# Autodesk Inventor assembly: 付け根_1
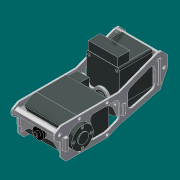
[picture p0: Inventor's stored thumbnail of the model, 180x180]
Saved by Autodesk Inventor 2016 (Build 200138000, 138)
## iProperties
Created: 2016-04-27
Part Number: 付け根_1
Document SubType Name: Assembly
Designer: hiroaki
Mass: 228.077 g
Surface Area: 379.105 cm^2
Volume: 115.513 cm^3
Density: 1.97447 g/cm^3
Author: hiroaki
## Documents named in this file (12)
- C:\Users\hiro\Documents\kenkyuu\二足\二足ver6.0\下半身\足首\足首_1.iam
- C:\Users\hiro\Documents\kenkyuu\二足\二足ver6.0\既製品\B3M11xx.ipt
- C:\Users\hiro\Documents\kenkyuu\二足\二足ver6.0\既製品\free_horn.ipt
- C:\Users\hiro\Documents\kenkyuu\二足\二足ver6.0\下半身\足首\足首_メインフレーム_1_1.ipt
- C:\Users\hiro\Documents\kenkyuu\二足\二足ver6.0\下半身\足首\足首_サブフレーム_1_1.ipt
- C:\Users\hiro\Documents\kenkyuu\二足\二足ver6.0\下半身\足首\足首_サブフレーム_1_2.ipt
- C:\Users\hiro\Documents\kenkyuu\二足\二足ver6.0\下半身\足首\足首_メインフレーム_1_1_MIR.ipt
- C:\Users\hiro\Documents\kenkyuu\二足\二足ver6.0\下半身\足首\足首_サブフレーム_1_3.ipt
- C:\Users\hiro\Documents\kenkyuu\二足\二足ver6.0\下半身\足裏\足裏_サブフレーム_1_2.ipt
- C:\Users\hiro\Documents\kenkyuu\二足\二足ver6.0\既製品\B3M10xx.ipt
- C:\Users\hiro\Documents\kenkyuu\二足\二足ver6.0\既製品\ASU-340.ipt
- C:\Users\hiro\Documents\kenkyuu\二足\二足ver6.0\既製品\CC-0311-08B.ipt
## Components (12 placed, 10 different names)
1. B3M11xx:1 — 挿入:23, 挿入:24, 挿入:25, 挿入:26, 挿入:27, 挿入:36, 挿入:37, 挿入:38, 挿入:39, メイト:7
2. free_horn:1 — 挿入:23
3. 足首_メインフレーム_1_1:1 — 挿入:24, 挿入:25, 挿入:26, 挿入:27, メイト:1, メイト:2, メイト:3, メイト:4, メイト:5, メイト:6, メイト:8, 挿入:46, 挿入:48, 角度:2
4. 足首_サブフレーム_1_1:1 — メイト:1, メイト:2, メイト:3, 挿入:42, 挿入:45
5. 足首_サブフレーム_1_2:1 — メイト:4, メイト:5, メイト:6, 挿入:43, 挿入:44
6. 足首_メインフレーム_1_1_MIR:1 — 挿入:36, 挿入:37, 挿入:38, 挿入:39, メイト:9, 挿入:47, 挿入:49, 角度:1
7. 足首_サブフレーム_1_3:1 — メイト:7, メイト:8, メイト:9, 挿入:51
8. 足裏_サブフレーム_1_2:1 — 挿入:50
9. B3M11xx:3 — 挿入:42, 挿入:43, 挿入:44, 挿入:45
10. ASU-340:1 — 挿入:46, 挿入:47, 角度:1
11. ASU-340:2 — 挿入:48, 挿入:49, 角度:2
12. CC-0311-08B:1 — 挿入:50, 挿入:51
## Relationships (30: Insert 19, Mate 9, Angle 2)
- 挿入:23 [Insert]: B3M11xx:1 ↔ free_horn:1
- 挿入:24 [Insert]: B3M11xx:1 ↔ 足首_メインフレーム_1_1:1
- 挿入:25 [Insert]: B3M11xx:1 ↔ 足首_メインフレーム_1_1:1
- 挿入:26 [Insert]: B3M11xx:1 ↔ 足首_メインフレーム_1_1:1
- 挿入:27 [Insert]: B3M11xx:1 ↔ 足首_メインフレーム_1_1:1
- メイト:1 [Mate] (0.025 mm): 足首_メインフレーム_1_1:1 ↔ 足首_サブフレーム_1_1:1
- メイト:2 [Mate]: 足首_メインフレーム_1_1:1 ↔ 足首_サブフレーム_1_1:1
- メイト:3 [Mate] (0.025 mm): 足首_メインフレーム_1_1:1 ↔ 足首_サブフレーム_1_1:1
- メイト:4 [Mate]: 足首_メインフレーム_1_1:1 ↔ 足首_サブフレーム_1_2:1
- メイト:5 [Mate] (0.025 mm): 足首_メインフレーム_1_1:1 ↔ 足首_サブフレーム_1_2:1
- メイト:6 [Mate] (0.025 mm): 足首_メインフレーム_1_1:1 ↔ 足首_サブフレーム_1_2:1
- 挿入:36 [Insert]: B3M11xx:1 ↔ 足首_メインフレーム_1_1_MIR:1
- 挿入:37 [Insert]: B3M11xx:1 ↔ 足首_メインフレーム_1_1_MIR:1
- 挿入:38 [Insert]: B3M11xx:1 ↔ 足首_メインフレーム_1_1_MIR:1
- 挿入:39 [Insert]: B3M11xx:1 ↔ 足首_メインフレーム_1_1_MIR:1
- メイト:7 [Mate]: B3M11xx:1 ↔ 足首_サブフレーム_1_3:1
- メイト:8 [Mate]: 足首_メインフレーム_1_1:1 ↔ 足首_サブフレーム_1_3:1
- メイト:9 [Mate] (0.025 mm): 足首_メインフレーム_1_1_MIR:1 ↔ 足首_サブフレーム_1_3:1
- 挿入:42 [Insert]: 足首_サブフレーム_1_1:1 ↔ B3M11xx:3
- 挿入:43 [Insert]: 足首_サブフレーム_1_2:1 ↔ B3M11xx:3
- 挿入:44 [Insert]: 足首_サブフレーム_1_2:1 ↔ B3M11xx:3
- 挿入:45 [Insert]: 足首_サブフレーム_1_1:1 ↔ B3M11xx:3
- 挿入:46 [Insert]: 足首_メインフレーム_1_1:1 ↔ ASU-340:1
- 挿入:47 [Insert]: 足首_メインフレーム_1_1_MIR:1 ↔ ASU-340:1
- 挿入:48 [Insert]: 足首_メインフレーム_1_1:1 ↔ ASU-340:2
- 挿入:49 [Insert]: 足首_メインフレーム_1_1_MIR:1 ↔ ASU-340:2
- 角度:1 [Angle] (0 deg): 足首_メインフレーム_1_1_MIR:1 ↔ ASU-340:1
- 角度:2 [Angle] (0 deg): 足首_メインフレーム_1_1:1 ↔ ASU-340:2
- 挿入:50 [Insert]: 足裏_サブフレーム_1_2:1 ↔ CC-0311-08B:1
- 挿入:51 [Insert]: 足首_サブフレーム_1_3:1 ↔ CC-0311-08B:1
